# Autodesk Inventor assembly: Assembly222222
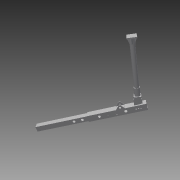
[picture p0: Inventor's stored thumbnail of the model, 180x180]
Saved by Autodesk Inventor 2014 SP2 (Build 180246200, 246)
## iProperties
Created: 2019-06-24
Part Number: Assembly222222
Document SubType Name: Assembly
Designer: USER PC
Author: USER PC
## Documents named in this file (6)
- C:\Users\USER PC\Desktop\United Tractors\New folder\Assembly222222.iam
- C:\Users\USER PC\Desktop\United Tractors\New folder\atas 1.ipt
- C:\Users\USER PC\Desktop\United Tractors\New folder\atas 2.ipt
- C:\Users\USER PC\Desktop\United Tractors\New folder\badan 1.ipt
- C:\Users\USER PC\Desktop\United Tractors\New folder\badan 2.ipt
- C:\Users\USER PC\Desktop\United Tractors\New folder\BADAN 3.ipt
## Components (5 placed, 5 different names)
1. badan 1:1 — Insert:1, Mate:2, Mate:4, Rigid:1, Rigid:2
2. badan 2:1 — Insert:1, Rigid:2
3. BADAN 3:1 — Mate:2, Mate:4, Rigid:1, Rigid:3
4. atas 1:1 — Rigid:3, Rotational:1
5. atas 2:1 — Rotational:1
## Relationships (7: WeldJoint 3, Mate 2, Insert 1, RevoluteJoint 1)
- Insert:1: badan 1:1 ↔ badan 2:1
- Mate:2: badan 1:1 ↔ BADAN 3:1
- Mate:4: badan 1:1 ↔ BADAN 3:1
- Rigid:1 [WeldJoint]: badan 1:1 ↔ BADAN 3:1
- Rigid:2 [WeldJoint]: badan 1:1 ↔ badan 2:1
- Rigid:3 [WeldJoint]: BADAN 3:1 ↔ atas 1:1
- Rotational:1 [RevoluteJoint]: atas 1:1 ↔ atas 2:1
